# Autodesk Inventor assembly: Crank_Slider_Fixer
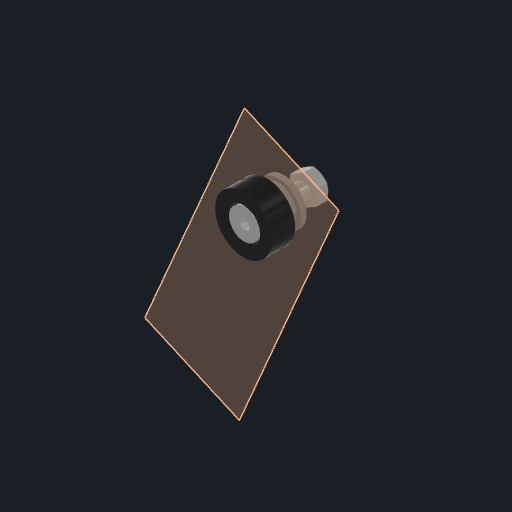
[picture p0: Inventor's stored thumbnail of the model, 512x512]
Saved by Autodesk Inventor 2024.3 (Build 283343000, 343)
## iProperties
Created: 2024-01-28
Part Number: Crank_Slider_Fixer
Document SubType Name: Assembly
Designer: 김대겸
Author: 김대겸
## Documents named in this file (6)
- C:\Users\ASUS\Desktop\test\v1_Frame\Crank_Slider_Fixer.iam
- C:\Users\ASUS\Desktop\test\v1_Frame\MISUMI\LED-0606.ipt
- C:\Users\ASUS\Desktop\test\v1_Frame\Handmade tiered cover_9mm_Wide.ipt
- C:\Users\ASUS\Desktop\test\v1_Frame\Ubber_Washer_1.5mm.ipt
- C:\Users\ASUS\Desktop\test\v1_Frame\MISUMI\CSHCS-SUSTBS-M4-20.ipt
- C:\Users\ASUS\Desktop\test\v1_Frame\MISUMI\SLBNR4.ipt
## Components (5 placed, 5 different names)
1. LED-0606:1 — 메이트:3
2. Handmade tiered cover_9mm_Wide:1 — 삽입:1
3. Ubber_Washer_1.5mm:1
4. CSHCS-SUSTBS-M4-20:1 — 삽입:1, 메이트:4
5. SLBNR4:1 — 메이트:3, 메이트:4
## Relationships (5: Mate 4, Insert 1)
- [Mate]: Handmade tiered cover_9mm_Wide:1 ↔ Ubber_Washer_1.5mm:1
- [Mate]: Handmade tiered cover_9mm_Wide:1 ↔ Ubber_Washer_1.5mm:1
- 삽입:1 [Insert]: Handmade tiered cover_9mm_Wide:1 ↔ CSHCS-SUSTBS-M4-20:1
- 메이트:3 [Mate] (5 mm): LED-0606:1 ↔ SLBNR4:1
- 메이트:4 [Mate]: CSHCS-SUSTBS-M4-20:1 ↔ SLBNR4:1
